# Autodesk Inventor assembly: 13 in^3 drivetrain
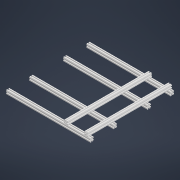
[picture p0: Inventor's stored thumbnail of the model, 180x180]
Saved by Autodesk Inventor 2022 (Build 260153000, 153)
## iProperties
Created: 2021-10-01
Part Number: 13 in^3 drivetrain
Document SubType Name: Assembly
Designer: izack
Author: izack
## Documents named in this file (2)
- E:\CAD Modeling\GithubCAD\ComputerAidedDesign\2021-22\FTC\#13822 Robovikes\Proof of Concept\13 in^3 drivetrain.iam
- E:\CAD Modeling\GithubCAD\ComputerAidedDesign\2021-22\FTC\#13822 Robovikes\Proof of Concept\15mm Extrusion - 330.2mm - 90° Ends.ipt
## Components (6 placed, 1 different names)
1. 15mm Extrusion - 330.2mm - 90° Ends:1 — Flush:1, Mate:1, Flush:2, Mate:2, Flush:5, Mate:6, Flush:7
2. 15mm Extrusion - 330.2mm - 90° Ends:2 — Flush:1, Mate:1, Flush:3, Mate:3
3. 15mm Extrusion - 330.2mm - 90° Ends:3 — Flush:2, Mate:2, Flush:4, Mate:5, Mate:7
4. 15mm Extrusion - 330.2mm - 90° Ends:4 — Mate:6, Flush:7, Mate:7
5. 15mm Extrusion - 330.2mm - 90° Ends:5 — Mate:4, Mate:5, Flush:6
6. 15mm Extrusion - 330.2mm - 90° Ends:6 — Flush:3, Flush:4, Mate:3, Flush:5, Mate:4, Flush:6
## Relationships (14: Flush 7, Mate 7)
- Flush:1: 15mm Extrusion - 330.2mm - 90° Ends:1 ↔ 15mm Extrusion - 330.2mm - 90° Ends:2
- Mate:1: 15mm Extrusion - 330.2mm - 90° Ends:1 ↔ 15mm Extrusion - 330.2mm - 90° Ends:2
- Flush:2: 15mm Extrusion - 330.2mm - 90° Ends:1 ↔ 15mm Extrusion - 330.2mm - 90° Ends:3
- Mate:2: 15mm Extrusion - 330.2mm - 90° Ends:1 ↔ 15mm Extrusion - 330.2mm - 90° Ends:3
- Flush:3: 15mm Extrusion - 330.2mm - 90° Ends:2 ↔ 15mm Extrusion - 330.2mm - 90° Ends:6
- Flush:4: 15mm Extrusion - 330.2mm - 90° Ends:3 ↔ 15mm Extrusion - 330.2mm - 90° Ends:6
- Mate:3: 15mm Extrusion - 330.2mm - 90° Ends:2 ↔ 15mm Extrusion - 330.2mm - 90° Ends:6
- Flush:5: 15mm Extrusion - 330.2mm - 90° Ends:1 ↔ 15mm Extrusion - 330.2mm - 90° Ends:6
- Mate:4 (76.2 mm): 15mm Extrusion - 330.2mm - 90° Ends:5 ↔ 15mm Extrusion - 330.2mm - 90° Ends:6
- Mate:5: 15mm Extrusion - 330.2mm - 90° Ends:3 ↔ 15mm Extrusion - 330.2mm - 90° Ends:5
- Flush:6: 15mm Extrusion - 330.2mm - 90° Ends:5 ↔ 15mm Extrusion - 330.2mm - 90° Ends:6
- Mate:6 (76.2 mm): 15mm Extrusion - 330.2mm - 90° Ends:1 ↔ 15mm Extrusion - 330.2mm - 90° Ends:4
- Flush:7: 15mm Extrusion - 330.2mm - 90° Ends:1 ↔ 15mm Extrusion - 330.2mm - 90° Ends:4
- Mate:7: 15mm Extrusion - 330.2mm - 90° Ends:3 ↔ 15mm Extrusion - 330.2mm - 90° Ends:4
